# Autodesk Inventor assembly: Montagem_MANIPULADOR
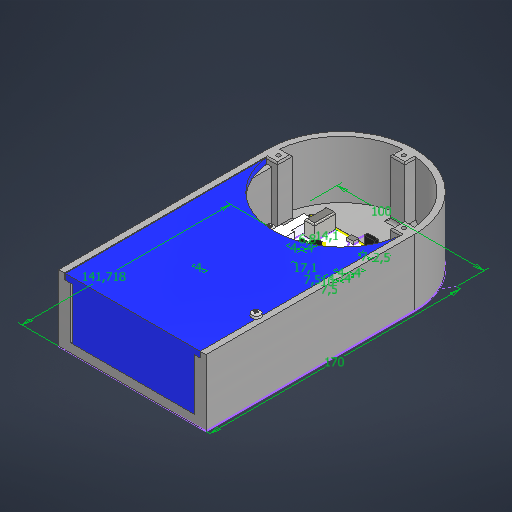
[picture p0: Inventor's stored thumbnail of the model, 512x512]
Saved by Autodesk Inventor 2027.1 (Build 311270010, 270A)
## iProperties
Created: 2026-08-16
Part Number: Montagem_MANIPULADOR
Document SubType Name: Assembly
Designer: Evellyn
Author: Evellyn
## Documents named in this file (5)
- C:\Users\Evellyn\Desktop\New-Robotic-Arm\mecanica\partes_ipt\Montagem_MANIPULADOR.iam
- C:\Users\Evellyn\Desktop\New-Robotic-Arm\mecanica\partes_ipt\BASE_MANIPULADOR.ipt
- C:\Users\Evellyn\Desktop\New-Robotic-Arm\mecanica\partes_ipt\MONTAGEM_BASE_ELETRONICA.iam
- C:\Users\Evellyn\Desktop\New-Robotic-Arm\mecanica\partes_ipt\TAMPA_BASE.ipt
- C:\Users\Evellyn\Documents\Inventor\Content Center Files\R2027\pt-BR\DIN 7985 (H)\DIN 7985 (H) - M3x6-H.ipt
## Components (8 placed, 4 different names)
1. BASE_MANIPULADOR:1 — Coincidente:1, Coincidente:2, Coincidente:3, Coincidente:4, Coincidente:5, Coincidente:6, Coincidente:9, Coincidente:15, Coincidente:16, Coincidente:17
2. MONTAGEM_BASE_ELETRONICA:1 [sub-assembly] — Coincidente:4, Coincidente:5, Coincidente:6, Coincidente:7, Coincidente:8, Coincidente:10, Coincidente:11, Coincidente:12, Coincidente:13, Coincidente:14
3. DIN 7985 (H) M3x6-H:1 — Coincidente:7, Coincidente:8
4. DIN 7985 (H) M3x6-H:2 — Coincidente:9, Coincidente:10
5. DIN 7985 (H) M3x6-H:3 — Coincidente:11, Coincidente:12
6. DIN 7985 (H) M3x6-H:4 — Coincidente:13, Coincidente:14
7. TAMPA_BASE:1 — Coincidente:15, Coincidente:16, Coincidente:17, Coincidente:18, Coincidente:19
8. DIN 7985 (H) M3x6-H:5 — Coincidente:18, Coincidente:19
## Relationships (19: Mate 19)
- Coincidente:1 [Mate]: BASE_MANIPULADOR:1
- Coincidente:2 [Mate]: BASE_MANIPULADOR:1
- Coincidente:3 [Mate]: BASE_MANIPULADOR:1
- Coincidente:4 [Mate]: BASE_MANIPULADOR:1 ↔ MONTAGEM_BASE_ELETRONICA:1
- Coincidente:5 [Mate]: BASE_MANIPULADOR:1 ↔ MONTAGEM_BASE_ELETRONICA:1
- Coincidente:6 [Mate]: BASE_MANIPULADOR:1 ↔ MONTAGEM_BASE_ELETRONICA:1
- Coincidente:7 [Mate]: MONTAGEM_BASE_ELETRONICA:1 ↔ DIN 7985 (H) M3x6-H:1
- Coincidente:8 [Mate]: MONTAGEM_BASE_ELETRONICA:1 ↔ DIN 7985 (H) M3x6-H:1
- Coincidente:9 [Mate]: BASE_MANIPULADOR:1 ↔ DIN 7985 (H) M3x6-H:2
- Coincidente:10 [Mate]: MONTAGEM_BASE_ELETRONICA:1 ↔ DIN 7985 (H) M3x6-H:2
- Coincidente:11 [Mate]: MONTAGEM_BASE_ELETRONICA:1 ↔ DIN 7985 (H) M3x6-H:3
- Coincidente:12 [Mate]: MONTAGEM_BASE_ELETRONICA:1 ↔ DIN 7985 (H) M3x6-H:3
- Coincidente:13 [Mate]: MONTAGEM_BASE_ELETRONICA:1 ↔ DIN 7985 (H) M3x6-H:4
- Coincidente:14 [Mate]: MONTAGEM_BASE_ELETRONICA:1 ↔ DIN 7985 (H) M3x6-H:4
- Coincidente:15 [Mate]: BASE_MANIPULADOR:1 ↔ TAMPA_BASE:1
- Coincidente:16 [Mate]: BASE_MANIPULADOR:1 ↔ TAMPA_BASE:1
- Coincidente:17 [Mate]: BASE_MANIPULADOR:1 ↔ TAMPA_BASE:1
- Coincidente:18 [Mate]: TAMPA_BASE:1 ↔ DIN 7985 (H) M3x6-H:5
- Coincidente:19 [Mate]: TAMPA_BASE:1 ↔ DIN 7985 (H) M3x6-H:5
